# Autodesk Inventor assembly: Elevator Sprocket with Sprockets_MIR
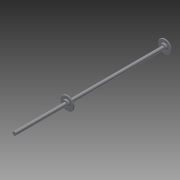
[picture p0: Inventor's stored thumbnail of the model, 180x180]
Saved by Autodesk Inventor 2015 (Build 190159000, 159)
## iProperties
Created: 2015-01-17
Part Number: Elevator Sprocket with Sprockets_MIR
Document SubType Name: Assembly
Designer: chapale16
Author: chapale16
## Documents named in this file (3)
- H:\Elevator Sprocket with Sprockets_MIR.iam
- H:\Elevator Axle_MIR1.ipt
- H:\Sprocket Large_MIR.ipt
## Components (3 placed, 2 different names)
1. Elevator Axle_MIR1:1 — Mate:2
2. Sprocket Large_MIR:1 — Flush:2
3. Sprocket Large_MIR:2 — Mate:2, Flush:2
## Relationships (2: Mate 1, Flush 1)
- Mate:2: Elevator Axle_MIR1:1 ↔ Sprocket Large_MIR:2
- Flush:2 (361.95 mm): Sprocket Large_MIR:1 ↔ Sprocket Large_MIR:2
